# Autodesk Inventor assembly: Knob Assembly
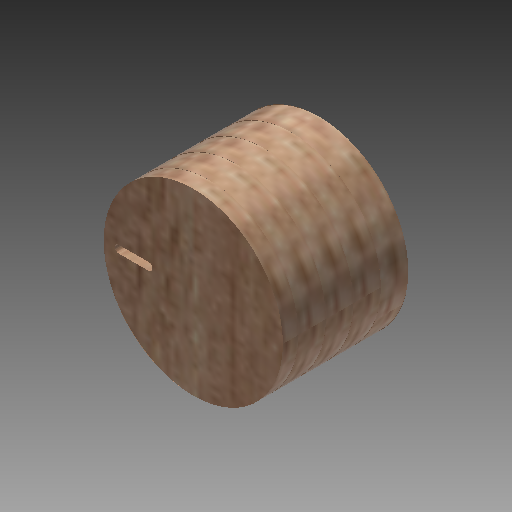
[picture p0: Inventor's stored thumbnail of the model, 512x512]
Saved by Autodesk Inventor 2018 (Build 220112000, 112)
## iProperties
Created: 2017-12-06
Part Number: Knob Assembly
Document SubType Name: Assembly
Designer: Andrew
Author: Andrew
## Documents named in this file (4)
- D:\Users\Andrew\OneDrive\3D Models\AM Radio\Knob Assembly.iam
- D:\Users\Andrew\OneDrive\3D Models\AM Radio\Knob.ipt
- D:\Users\Andrew\OneDrive\3D Models\AM Radio\KnobCover.ipt
- D:\Users\Andrew\OneDrive\3D Models\AM Radio\KnobSpacer.ipt
## Components (5 placed, 3 different names)
1. Knob:1 — Flush:4, Flush:5, Mate:1, Mate:2, Mate:4, Flush:6
2. KnobCover:1 — Flush:1, Flush:2, Flush:3, Flush:4, Flush:5, Mate:1
3. KnobSpacer:1 — Mate:3, Mate:5, Mate:6, Mate:7
4. Knob:2 — Mate:2, Mate:3, Mate:4, Mate:5, Flush:6
5. KnobSpacer:2 — Mate:6, Mate:7
## Relationships (13: Mate 7, Flush 6)
- Flush:1: KnobCover:1
- Flush:2: KnobCover:1
- Flush:3: KnobCover:1
- Flush:4: Knob:1 ↔ KnobCover:1
- Flush:5: Knob:1 ↔ KnobCover:1
- Mate:1: Knob:1 ↔ KnobCover:1
- Mate:2: Knob:1 ↔ Knob:2
- Mate:3: KnobSpacer:1 ↔ Knob:2
- Mate:4: Knob:1 ↔ Knob:2
- Mate:5: KnobSpacer:1 ↔ Knob:2
- Flush:6: Knob:1 ↔ Knob:2
- Mate:6: KnobSpacer:1 ↔ KnobSpacer:2
- Mate:7: KnobSpacer:1 ↔ KnobSpacer:2
